# Autodesk Inventor assembly: disk
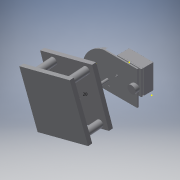
[picture p0: Inventor's stored thumbnail of the model, 180x180]
Saved by Autodesk Inventor 2019 (Build 230136000, 136)
## iProperties
Created: 2020-02-20
Part Number: disk
Document SubType Name: Assembly
Designer: ADMIN
Author: ADMIN
## Documents named in this file (10)
- C:\Users\ADMIN\Desktop\EXPLORATION\expo\final1.0023.iam
- C:\Users\ADMIN\Desktop\EXPLORATION\expo\holder.ipt
- C:\Users\ADMIN\Desktop\EXPLORATION\expo\glassplane.ipt
- C:\Users\ADMIN\Desktop\EXPLORATION\expo\rod.ipt
- C:\Users\ADMIN\Desktop\EXPLORATION\expo\wheel.ipt
- C:\Users\ADMIN\Desktop\EXPLORATION\expo\base1.ipt
- C:\Users\ADMIN\Desktop\EXPLORATION\expo\lowerbase.ipt
- C:\Users\ADMIN\Desktop\EXPLORATION\expo\stepper.ipt
- C:\Users\ADMIN\Desktop\EXPLORATION\expo\angle.ipt
- C:\Users\ADMIN\Desktop\EXPLORATION\expo\led.ipt
## Components (9 placed, 9 different names)
1. holder:1
2. glassplane:1
3. rod:1 — Mate:1, Mate:2
4. wheel:1 — Mate:1
5. base1:1 — Mate:2
6. lowerbase:1
7. stepper:1
8. angle:1
9. led:2
## Relationships (2: Mate 2)
- Mate:1: rod:1 ↔ wheel:1
- Mate:2: rod:1 ↔ base1:1
